# Autodesk Inventor assembly: X_CarriageR_V2_0
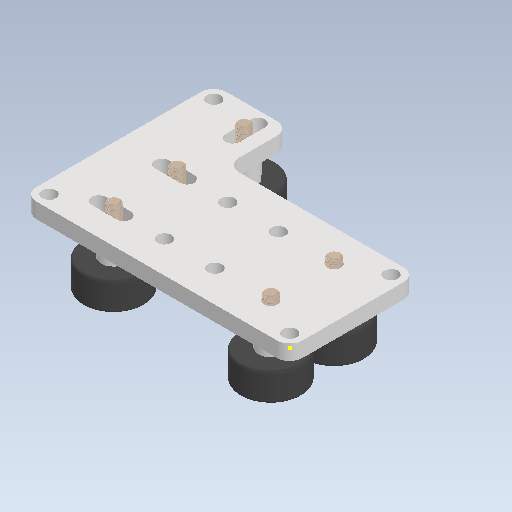
[picture p0: Inventor's stored thumbnail of the model, 512x512]
Saved by Autodesk Inventor 2021 (Build 250183000, 183)
## iProperties
Created: 2021-06-13
Part Number: X_CarriageR_V2_0
Document SubType Name: Assembly
Designer: Jorian Brusind
Author: Jorian Brusind
## Documents named in this file (5)
- C:\Users\Jorian Brusind\Documents\GitHub\PersonalProjects\HyperRail\Inventor Files\X_CarriageR_V2_0.iam
- C:\Users\Jorian Brusind\Documents\GitHub\PersonalProjects\HyperRail\Inventor Files\X_Carriage_Plate.ipt
- C:\Users\Jorian Brusind\Documents\GitHub\PersonalProjects\HyperRail\Inventor Files\11mm_BearingWheel.ipt
- C:\Users\Jorian Brusind\Documents\GitHub\PersonalProjects\HyperRail\Inventor Files\6mm_Spacer.ipt
- C:\Users\Jorian Brusind\Documents\GitHub\PersonalProjects\Inventor Projects\Useful models\Metric bolt\Bolt M5 30mm.ipt
## Components (16 placed, 4 different names)
1. X_Carriage_Plate:1 — Mate:1, Mate:2, Mate:3, Mate:5, Mate:7, Mate:8, Mate:9, Mate:10, Mate:12, Mate:14, Mate:16, Mate:18, Mate:20
2. 11mm_BearingWheel:1 — Mate:1, Mate:6, Flush:2, Mate:17, Mate:24
3. 11mm_BearingWheel:2 — Mate:5, Mate:6, Flush:1, Mate:11, Mate:21
4. 11mm_BearingWheel:3 — Mate:3, Mate:4, Flush:1, Flush:3, Mate:13, Mate:22, Mate:26
5. 11mm_BearingWheel:4 — Mate:2, Mate:4, Flush:2, Flush:3, Mate:7, Mate:19, Mate:25
6. 11mm_BearingWheel:5 — Mate:8, Mate:9, Mate:10, Mate:15, Mate:23
7. 6mm_Spacer:1 — Mate:19, Mate:20
8. 6mm_Spacer:2 — Mate:15, Mate:16
9. 6mm_Spacer:3 — Mate:17, Mate:18
10. 6mm_Spacer:4 — Mate:13, Mate:14
11. 6mm_Spacer:5 — Mate:11, Mate:12
12. Bolt M5 30mm:1 — Mate:24, Flush:4
13. Bolt M5 30mm:2 — Mate:25, Flush:7
14. Bolt M5 30mm:3 — Mate:23, Flush:6
15. Bolt M5 30mm:4 — Mate:21, Flush:4, Flush:5, Flush:6, Flush:7, Mate:26
16. Bolt M5 30mm:5 — Mate:22, Flush:5
## Relationships (33: Mate 26, Flush 7)
- Mate:1: X_Carriage_Plate:1 ↔ 11mm_BearingWheel:1
- Mate:2: X_Carriage_Plate:1 ↔ 11mm_BearingWheel:4
- Mate:3 (2.75 mm): X_Carriage_Plate:1 ↔ 11mm_BearingWheel:3
- Mate:4 (62 mm): 11mm_BearingWheel:3 ↔ 11mm_BearingWheel:4
- Mate:5 (2.75 mm): X_Carriage_Plate:1 ↔ 11mm_BearingWheel:2
- Mate:6 (62 mm): 11mm_BearingWheel:1 ↔ 11mm_BearingWheel:2
- Flush:1: 11mm_BearingWheel:2 ↔ 11mm_BearingWheel:3
- Flush:2: 11mm_BearingWheel:1 ↔ 11mm_BearingWheel:4
- Flush:3: 11mm_BearingWheel:3 ↔ 11mm_BearingWheel:4
- Mate:7 (-27 mm): X_Carriage_Plate:1 ↔ 11mm_BearingWheel:4
- Mate:8 (2.75 mm): X_Carriage_Plate:1 ↔ 11mm_BearingWheel:5
- Mate:9 (-10 mm): X_Carriage_Plate:1 ↔ 11mm_BearingWheel:5
- Mate:10 (-27 mm): X_Carriage_Plate:1 ↔ 11mm_BearingWheel:5
- Mate:11: 11mm_BearingWheel:2 ↔ 6mm_Spacer:5
- Mate:12: X_Carriage_Plate:1 ↔ 6mm_Spacer:5
- Mate:13: 11mm_BearingWheel:3 ↔ 6mm_Spacer:4
- Mate:14: X_Carriage_Plate:1 ↔ 6mm_Spacer:4
- Mate:15: 11mm_BearingWheel:5 ↔ 6mm_Spacer:2
- Mate:16: X_Carriage_Plate:1 ↔ 6mm_Spacer:2
- Mate:17: 11mm_BearingWheel:1 ↔ 6mm_Spacer:3
- Mate:18: X_Carriage_Plate:1 ↔ 6mm_Spacer:3
- Mate:19: 11mm_BearingWheel:4 ↔ 6mm_Spacer:1
- Mate:20: X_Carriage_Plate:1 ↔ 6mm_Spacer:1
- Mate:21: 11mm_BearingWheel:2 ↔ Bolt M5 30mm:4
- Mate:22: 11mm_BearingWheel:3 ↔ Bolt M5 30mm:5
- Mate:23: 11mm_BearingWheel:5 ↔ Bolt M5 30mm:3
- Mate:24: 11mm_BearingWheel:1 ↔ Bolt M5 30mm:1
- Mate:25: 11mm_BearingWheel:4 ↔ Bolt M5 30mm:2
- Flush:4: Bolt M5 30mm:1 ↔ Bolt M5 30mm:4
- Flush:5: Bolt M5 30mm:4 ↔ Bolt M5 30mm:5
- Flush:6: Bolt M5 30mm:3 ↔ Bolt M5 30mm:4
- Flush:7: Bolt M5 30mm:2 ↔ Bolt M5 30mm:4
- Mate:26: 11mm_BearingWheel:3 ↔ Bolt M5 30mm:4
